# Autodesk Inventor assembly: Stewart Platform
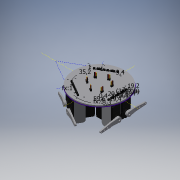
[picture p0: Inventor's stored thumbnail of the model, 180x180]
Saved by Autodesk Inventor 2018.2 (Build 222227000, 227)
## iProperties
Created: 2018-02-17
Part Number: Stewart Platform
Material: Generisch
Document SubType Name: Assembly
Designer: JochenAlt
Author: JochenAlt
## Documents named in this file (3)
- D:\Projects\PrivateDancer\CAD\Stewart Platform-Innenanordnung.iam
- D:\Projects\PrivateDancer\CAD\ServoHolder.iam
- D:\Projects\PrivateDancer\CAD\Stewart-Platform-Base-Innenanordnung.ipt
## Components (4 placed, 2 different names)
1. ServoHolder:1 [sub-assembly] — Passend:5, Passend:6
2. ServoHolder:2 [sub-assembly] — Passend:3, Passend:4
3. ServoHolder:3 [sub-assembly] — Passend:1, Passend:2
4. Stewart-Platform-Base:1 — Passend:1, Passend:2, Passend:3, Passend:4, Passend:5, Passend:6
## Relationships (6: Mate 6)
- Passend:1 [Mate]: ServoHolder:3 ↔ Stewart-Platform-Base:1
- Passend:2 [Mate]: ServoHolder:3 ↔ Stewart-Platform-Base:1
- Passend:3 [Mate]: ServoHolder:2 ↔ Stewart-Platform-Base:1
- Passend:4 [Mate]: ServoHolder:2 ↔ Stewart-Platform-Base:1
- Passend:5 [Mate]: ServoHolder:1 ↔ Stewart-Platform-Base:1
- Passend:6 [Mate]: ServoHolder:1 ↔ Stewart-Platform-Base:1
